# Autodesk Inventor assembly: Head2
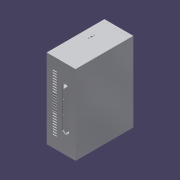
[picture p0: Inventor's stored thumbnail of the model, 180x180]
Saved by Autodesk Inventor 2017 SP1 (Build 210196100, 196)
## iProperties
Created: 2018-06-14
Part Number: Head2
Document SubType Name: Assembly
Designer: Zach
Author: Zach
## Documents named in this file (2)
- C:\Users\Zach\Documents\GitHub\tr1_description\meshes\Visual Assembly\Head.iam
- C:\Users\Zach\slaterobots.com\Slate Robotics OneDrive - Documents\CodyM\Head.ipt
## Components (1 placed, 1 different names)
1. Head:2 — Mate:3, Flush:1, Angle:2
## Relationships (3: Mate 1, Flush 1, Angle 1)
- Mate:3: Head:2
- Flush:1 (137.5 mm): Head:2
- Angle:2 (0 deg): Head:2
